# Autodesk Inventor assembly: slider
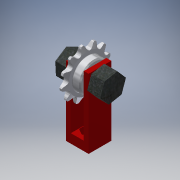
[picture p0: Inventor's stored thumbnail of the model, 180x180]
Saved by Autodesk Inventor 2016 (Build 200138000, 138)
## iProperties
Created: 2016-01-17
Part Number: slider
Document SubType Name: Assembly
Designer: gus
Mass: 90.937 g
Surface Area: 129.496 cm^2
Volume: 23.2302 cm^3
Density: 3.91459 g/cm^3
Author: gus
## Documents named in this file (5)
- \\Mac\Home\Desktop\2016 robot cad\chassis\chain tensioner\slider.iam
- \\Mac\Home\Desktop\2016 robot cad\chassis\chain tensioner\217-2662-STEP-20140807.ipt
- \\Mac\Home\Desktop\2016 robot cad\chassis\chain tensioner\half-inch hex nut.ipt
- \\Mac\Home\Desktop\2016 robot cad\chassis\chain tensioner\short half-inch hex bolt.ipt
- \\Mac\Home\Desktop\2016 robot cad\chassis\chain tensioner\silider shaft.ipt
## Components (4 placed, 4 different names)
1. 217-2662-STEP-20140807:1 — Rotational:3
2. half-inch hex nut:1 — Rotational:2
3. short half-inch hex bolt:1 — Rotational:1
4. silider shaft:1 — Rotational:1, Rotational:2, Rotational:3
## Relationships (3: RevoluteJoint 3)
- Rotational:1 [RevoluteJoint]: short half-inch hex bolt:1 ↔ silider shaft:1
- Rotational:2 [RevoluteJoint]: half-inch hex nut:1 ↔ silider shaft:1
- Rotational:3 [RevoluteJoint]: 217-2662-STEP-20140807:1 ↔ silider shaft:1
